# Autodesk Inventor assembly: Samenstelling Frame 2.3
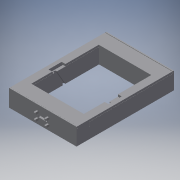
[picture p0: Inventor's stored thumbnail of the model, 180x180]
Saved by Autodesk Inventor 2018.3 (Build 223284000, 284)
## iProperties
Created: 2020-12-10
Part Number: Samenstelling Frame 2.3
Document SubType Name: Assembly
Designer: daanv
Author: daanv
## Documents named in this file (3)
- C:\Users\daanv\OneDrive\Documenten\Life\Avans Project RED\Gebouw\Samenstelling Frame 2.3.iam
- C:\Users\daanv\OneDrive\Documenten\Life\Avans Project RED\Gebouw\Bovenplaat Frame 2.3.ipt
- C:\Users\daanv\OneDrive\Documenten\Life\Avans Project RED\Gebouw\Frame V2.3.ipt
## Components (2 placed, 2 different names)
1. Bovenplaat Frame 2.3:1 — Mate:1, Mate:2
2. Frame V2.3:1 — Mate:1, Mate:2
## Relationships (2: Mate 2)
- Mate:1: Bovenplaat Frame 2.3:1 ↔ Frame V2.3:1
- Mate:2: Bovenplaat Frame 2.3:1 ↔ Frame V2.3:1
